# Autodesk Inventor assembly: RioAndStands
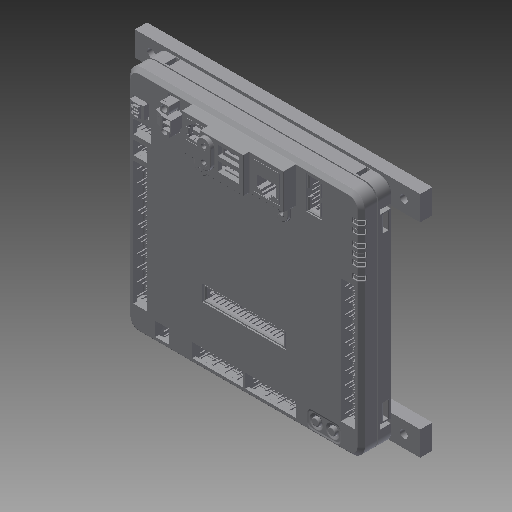
[picture p0: Inventor's stored thumbnail of the model, 512x512]
Saved by Autodesk Inventor 2019 (Build 230136000, 136)
## iProperties
Created: 2020-03-03
Part Number: RioAndStands
Document SubType Name: Assembly
Designer: james
Author: james
## Documents named in this file (3)
- F:\JimsRobot\FIRSTRobots\Design\Library\Jims\RioAndStands.iam
- F:\JimsRobot\FIRSTRobots\Design\Library\Jims\RioConnectors.ipt
- F:\JimsRobot\FIRSTRobots\Design\Library\AndyMark\roboRIO CAD\3d\cd_roborio.ipt
## Components (3 placed, 2 different names)
1. RioConnectors:1 — Mate:1, Mate:3, Mate:4
2. RioConnectors:2 — Mate:2, Mate:5, Mate:6
3. cd_roborio:1 — Mate:1, Mate:2, Mate:3, Mate:4, Mate:5, Mate:6
## Relationships (6: Mate 6)
- Mate:1: RioConnectors:1 ↔ cd_roborio:1
- Mate:2: RioConnectors:2 ↔ cd_roborio:1
- Mate:3: RioConnectors:1 ↔ cd_roborio:1
- Mate:4: RioConnectors:1 ↔ cd_roborio:1
- Mate:5: RioConnectors:2 ↔ cd_roborio:1
- Mate:6: RioConnectors:2 ↔ cd_roborio:1
